# Autodesk Inventor assembly: A2017_T2_05
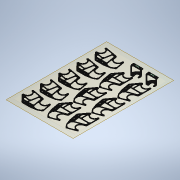
[picture p0: Inventor's stored thumbnail of the model, 180x180]
Saved by Autodesk Inventor 2022 (Build 260153000, 153)
## iProperties
Created: 2022-09-28
Part Number: A2017_T2_05
Document SubType Name: Assembly
Designer: Masato
Author: Masato
## Documents named in this file (4)
- C:\Users\ヨコオリク\Documents\CITBrains\SUSTAINA-OP\Cam\A2017_T2\A2017_T2_05.iam
- C:\Users\ヨコオリク\Documents\CITBrains\SUSTAINA-OP\Cam\DisposableBoard.ipt
- C:\Users\ヨコオリク\Documents\CITBrains\SUSTAINA-OP\LowerBody\Knee\Knee_side_frame.ipt
- C:\Users\ヨコオリク\Documents\CITBrains\SUSTAINA-OP\UpperBody\Arm\Shoulder_side_frame.ipt
## Components (14 placed, 3 different names)
1. DisposableBoard:1 — フラッシュ:1, フラッシュ:2, フラッシュ:3, フラッシュ:4, フラッシュ:5, 正接:1, フラッシュ:6, 正接:2, フラッシュ:7, 正接:3
2. Knee_side_frame:1 — メイト:1, フラッシュ:5, 正接:1
3. Knee_side_frame:2
4. Knee_side_frame:3
5. Knee_side_frame:4
6. Knee_side_frame:5
7. Knee_side_frame:6 — メイト:2, フラッシュ:6, 正接:2
8. Knee_side_frame:7
9. Knee_side_frame:8
10. Knee_side_frame:9
11. Knee_side_frame:10
12. Knee_side_frame:11
13. Shoulder_side_frame:1 — メイト:3, フラッシュ:7, 正接:3
14. Shoulder_side_frame:2
## Component patterns: (5 elements, first: Knee_side_frame:1), (6 elements, first: Knee_side_frame:6), (2 elements, first: Shoulder_side_frame:1)
## Relationships (13: Flush 7, Mate 3, Tangent 3)
- フラッシュ:1 [Flush]: DisposableBoard:1
- フラッシュ:2 [Flush]: DisposableBoard:1
- フラッシュ:3 [Flush]: DisposableBoard:1
- フラッシュ:4 [Flush]: DisposableBoard:1
- メイト:1 [Mate]: Knee_side_frame:1
- フラッシュ:5 [Flush] (2.1 mm): DisposableBoard:1 ↔ Knee_side_frame:1
- 正接:1 [Tangent] (2.1 mm): DisposableBoard:1 ↔ Knee_side_frame:1
- メイト:2 [Mate]: Knee_side_frame:6
- フラッシュ:6 [Flush] (-2.1 mm): DisposableBoard:1 ↔ Knee_side_frame:6
- 正接:2 [Tangent] (2.1 mm): DisposableBoard:1 ↔ Knee_side_frame:6
- メイト:3 [Mate]: Shoulder_side_frame:1
- フラッシュ:7 [Flush] (-2.5 mm): DisposableBoard:1 ↔ Shoulder_side_frame:1
- 正接:3 [Tangent] (2 mm): DisposableBoard:1 ↔ Shoulder_side_frame:1
